# Autodesk Inventor assembly: ASY ДМФ 0100 Барабан v2.1
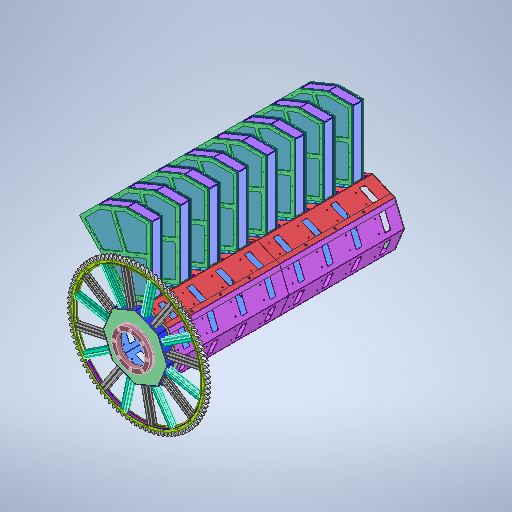
[picture p0: Inventor's stored thumbnail of the model, 512x512]
Saved by Autodesk Inventor 2025 (Build 290162010, 162A)
## iProperties
Created: 2024-04-28
Part Number: ASY ДМФ 0100 Барабан v2.1
Document SubType Name: Assembly
Designer: pokla
Author: pokla
## Documents named in this file (29)
- C:\Users\pokla\Documents\Inventor\ДФО\ДМФ\DMF-Disk-Micro-Filter\Барабан v2.1\ASY ДМФ 0100 Барабан v2.1.iam
- C:\Users\pokla\Documents\Inventor\ДФО\ДМФ\DMF-Disk-Micro-Filter\Барабан v2.1\DMF 01 21 Барабан торец НОС v2.1.ipt
- C:\Users\pokla\Documents\Inventor\ДФО\ДМФ\DMF-Disk-Micro-Filter\Барабан v2.1\DMF 01 13 Барабан Лист лев брт v2.1.ipt
- C:\Users\pokla\Documents\Inventor\ДФО\ДМФ\DMF-Disk-Micro-Filter\Барабан v2.1\DMF 01 14 Барабан Лист прав брт v2.1.ipt
- C:\Users\pokla\Documents\Inventor\ДФО\ДМФ\DMF-Disk-Micro-Filter\Барабан v2.1\DMF 01 31 Барабан Опорное кольцо НОС v2.1.ipt
- C:\Users\pokla\Documents\Inventor\ДФО\ДМФ\DMF-Disk-Micro-Filter\Барабан v2.1\DMF 01 17 опора крышки v2.1.ipt
- C:\Users\pokla\Documents\Inventor\ДФО\ДМФ\DMF-Disk-Micro-Filter\Барабан v2.1\DMF 000 размеры v2.1.ipt
- C:\Users\pokla\Documents\Inventor\ДФО\ДМФ\DMF-Disk-Micro-Filter\Барабан v2.1\DMF 01 12 Барабан усилитель v2.1.ipt
- C:\Users\pokla\Documents\Inventor\ДФО\ДМФ\DMF-Disk-Micro-Filter\Барабан v2.1\ASY DMF 010 cap v2.1.iam
- C:\Users\pokla\Documents\Inventor\ДФО\ДМФ\DMF-Disk-Micro-Filter\Барабан v2.1\DMF 01 32 Барабан Опорное кольцо КОРМА v2.1.ipt
- C:\Users\pokla\Documents\Inventor\ДФО\ДМФ\DMF-Disk-Micro-Filter\Барабан v2.1\DMF 01 22 Барабан торец КОРМА v2.1.ipt
- C:\Users\pokla\Documents\Inventor\ДФО\ДМФ\DMF-Disk-Micro-Filter\Барабан v2.1\ASY DMF filter package v2.1.iam
- C:\Users\pokla\Documents\Inventor\ДФО\ДМФ\DMF-Disk-Micro-Filter\Барабан v2.1\DMF 01 21 cylinder butt end nose.ipt
- C:\Users\pokla\Documents\Inventor\ДФО\ДМФ\DMF-Disk-Micro-Filter\Барабан v2.1\DMF 2.1 01 42 Gear way 2.ipt
- C:\Users\pokla\Documents\Inventor\ДФО\ДМФ\DMF-Disk-Micro-Filter\Барабан v2.1\DMF 2.1 01 43 Gear rim 3.ipt
- C:\Users\pokla\Documents\Inventor\ДФО\ДМФ\DMF-Disk-Micro-Filter\Барабан v2.1\DMF 2.1 01 44 Gear rim 4.ipt
- C:\Users\pokla\Documents\Inventor\ДФО\ДМФ\DMF-Disk-Micro-Filter\Барабан v2.1\DMF 2.1 01 45 Gear ring 5.ipt
- C:\Users\pokla\Documents\Inventor\ДФО\ДМФ\DMF-Disk-Micro-Filter\Барабан v2.1\DMF 2.1 01 46 Gear axis wheel 6.ipt
- C:\Users\pokla\Documents\Inventor\ДФО\ДМФ\DMF-Disk-Micro-Filter\Барабан v2.1\DMF 01 13 Барабан усилитель v2.1.ipt
- C:\Users\pokla\Documents\Inventor\ДФО\ДМФ\DMF-Disk-Micro-Filter\шестерни 06.09.2025\DMF sector big gear 2.1.ipt
- C:\Users\pokla\Documents\Inventor\ДФО\ДМФ\DMF-Disk-Micro-Filter\Барабан v2.1\DMF 01 15 drum sheet 1.ipt
- C:\Users\pokla\Documents\Inventor\ДФО\ДМФ\DMF-Disk-Micro-Filter\ДМФ 01 12 Барабан усилитель.ipt
- C:\Users\pokla\Documents\Inventor\ДФО\ДМФ\DMF-Disk-Micro-Filter\ДМФ 01 15 Барабан усилитель борта.ipt
- C:\Users\pokla\Documents\Inventor\ДФО\ДМФ\DMF-Disk-Micro-Filter\Барабан v2.1\DMF 2.1 Пластина паза маленькая.ipt
- C:\Users\pokla\Documents\Inventor\ДФО\ДМФ\DMF-Disk-Micro-Filter\Барабан v2.1\DMF 2.1 Пластина паза большая.ipt
- C:\Users\pokla\Documents\Inventor\ДФО\ДМФ\DMF-Disk-Micro-Filter\Барабан v2.1\DMF 01 14 Барабан Лист прав брт №2 v2.1.ipt
- C:\Users\pokla\Documents\Inventor\ДФО\ДМФ\DMF-Disk-Micro-Filter\Барабан v2.1\DMF 01 13 Барабан Лист лев брт №2 v2.1.ipt
- C:\Users\pokla\Documents\Inventor\ДФО\ДМФ\DMF-Disk-Micro-Filter\Барабан v2.1\ASY DMF 010 cap №2 v2.1.iam
- C:\Users\pokla\Documents\Inventor\ДФО\ДМФ\DMF-Disk-Micro-Filter\Барабан v2.1\DMF 01 17 опора крышки v2.1_CPY.ipt
## Components (125 placed, 36 different names)
1. DMF 000 размеры v2.1.ipt:1
2. DMF 01 21 Барабан торец НОС v2.1.ipt:1 — Mate:41, Flush:29, Flush:30, Mate:42, Flush:31, Flush:32, Rigid:80, Rigid:81
3. DMF 01 31 Барабан Опорное кольцо НОС v2.1.ipt:1 — Rigid:80
4. DMF 01 32 Барабан Опорное кольцо КОРМА v2.1.ipt:1 — Rigid:20
5. DMF 01 22 Барабан торец КОРМА v2.1.ipt:1 — Rigid:20, Rigid:51, Rigid:53, Mate:36, Flush:22, Flush:23, Mate:37, Flush:24, Flush:25, Mate:45, Flush:34, Flush:35
6. DMF 01 13 Барабан Лист лев брт v2.1.ipt:1 — Rigid:51, Rigid:86
7. DMF 01 14 Барабан Лист прав брт v2.1.ipt:1 — Rigid:53, Rigid:85
8. DMF 01 17 опора крышки v2.1.ipt:1 — Mate:37, Flush:24, Flush:25, Rigid:93
9. DMF 01 17 опора крышки v2.1.ipt:2 — Mate:36, Flush:22, Flush:23, Rigid:92
10. ASY DMF 010 cap v2.1.iam:1 [sub-assembly] — Mate:45, Flush:34, Flush:35, Rigid:84, Rigid:90, Rigid:91
11. DMF 01 21 cylinder butt end nose.ipt:1
12. DMF 2.1 01 45 Gear ring 5.ipt:1
13. DMF 2.1 01 46 Gear axis wheel 6.ipt:1
14. DMF 2.1 01 44 Gear rim 4.ipt:1 — Rigid:39, Rigid:40, Rigid:41
15. DMF 2.1 01 43 Gear rim 3.ipt:2 — Rigid:24, Rigid:35
16. DMF 2.1 01 43 Gear rim 3.ipt:1 — Rigid:24
17. DMF 2.1 01 43 Gear rim 3.ipt:3 — Rigid:35, Rigid:36, Rigid:39
18. DMF 2.1 01 43 Gear rim 3.ipt:4
19. DMF 2.1 01 43 Gear rim 3.ipt:5 — Rigid:36, Rigid:38, Rigid:81
20. DMF 2.1 01 43 Gear rim 3.ipt:6 — Rigid:42
21. DMF 2.1 01 43 Gear rim 3.ipt:7 — Rigid:38, Tangent:1
22. DMF 2.1 01 43 Gear rim 3.ipt:8
23. DMF 2.1 01 44 Gear rim 4.ipt:2 — Rigid:40
24. DMF 2.1 01 44 Gear rim 4.ipt:3 — Rigid:41
25. DMF 01 15 drum sheet 1.ipt:1 — Mate:41, Flush:29, Flush:30, Flush:33, Mate:43, Mate:50, Mate:51, Flush:38, Flush:39
26. DMF 01 15 drum sheet 1.ipt:2 — Mate:42, Flush:31, Flush:32, Mate:44
27. ДМФ 01 12 Барабан усилитель.ipt:2 — Rigid:56, Rigid:57, Flush:33, Mate:43, Mate:44, Rigid:89
28. ДМФ 01 15 Барабан усилитель борта.ipt:3 — Rigid:56
29. ДМФ 01 15 Барабан усилитель борта.ipt:4 — Rigid:57
30. DMF 01 14 Барабан Лист прав брт №2 v2.1:1 — Rigid:85
31. DMF 01 13 Барабан Лист лев брт №2 v2.1:1 — Rigid:86
32. ASY DMF 010 cap №2 v2.1:1 [sub-assembly] — Rigid:84, Flush:40, Mate:52, Mate:53
33. ДМФ 01 12 Барабан усилитель:3 — Flush:40, Mate:52, Mate:53, Rigid:89
34. ДМФ 01 15 Барабан усилитель борта:5
35. ДМФ 01 15 Барабан усилитель борта:6
36. DMF 01 17 опора крышки №2 v2.1:1 — Rigid:92
37. DMF 01 17 опора крышки №2 v2.1:2 — Rigid:93
38. DMF sector big gear 2.1.ipt:1 — Rigid:42
39. DMF sector big gear 2.1:2
40. DMF sector big gear 2.1:3
41. DMF sector big gear 2.1:4
42. DMF sector big gear 2.1:5
43. DMF sector big gear 2.1:6
44. DMF sector big gear 2.1:7
45. DMF sector big gear 2.1:8
46. DMF sector big gear 2.1:9
47. DMF sector big gear 2.1:10
48. DMF sector big gear 2.1:11
49. DMF sector big gear 2.1:12
50. DMF sector big gear 2.1:13
51. DMF sector big gear 2.1:14
52. DMF sector big gear 2.1:15
53. DMF sector big gear 2.1:16
54. DMF sector big gear 2.1:17
55. DMF sector big gear 2.1:18
56. DMF sector big gear 2.1:19
57. DMF sector big gear 2.1:20
58. DMF sector big gear 2.1:21
59. DMF sector big gear 2.1:22
60. DMF sector big gear 2.1:23
61. DMF sector big gear 2.1:24
62. DMF 01 13 Барабан усилитель v2.1.ipt:2 — Rigid:83, Tangent:1
63. DMF 01 12 Барабан усилитель v2.1.ipt:2 — Rigid:83, Symmetry:1, Mate:50, Flush:38
64. DMF 01 13 Барабан усилитель v2.1.ipt:1 — Rigid:82
65. DMF 01 12 Барабан усилитель v2.1.ipt:1 — Rigid:82, Symmetry:1, Mate:51, Flush:39
66. ДМФ 01 13 Барабан усилитель v2.0:3
67. DMF 01 12 Барабан усилитель v2.1:52
68. ДМФ 01 13 Барабан усилитель v2.0:4
69. DMF 01 12 Барабан усилитель v2.1:53
70. ДМФ 01 13 Барабан усилитель v2.0:5
71. DMF 01 12 Барабан усилитель v2.1:54
72. ДМФ 01 13 Барабан усилитель v2.0:6
73. DMF 01 12 Барабан усилитель v2.1:55
74. ДМФ 01 13 Барабан усилитель v2.0:7
75. DMF 01 12 Барабан усилитель v2.1:56
76. ДМФ 01 13 Барабан усилитель v2.0:8
77. DMF 01 12 Барабан усилитель v2.1:57
78. ДМФ 01 13 Барабан усилитель v2.0:9
79. DMF 01 12 Барабан усилитель v2.1:58
80. ДМФ 01 13 Барабан усилитель v2.0:10
81. DMF 01 12 Барабан усилитель v2.1:59
82. ДМФ 01 13 Барабан усилитель v2.0:11
83. DMF 01 12 Барабан усилитель v2.1:60
84. ДМФ 01 13 Барабан усилитель v2.0:12
85. DMF 01 12 Барабан усилитель v2.1:61
86. ДМФ 01 13 Барабан усилитель v2.0:13
87. DMF 01 12 Барабан усилитель v2.1:62
88. ДМФ 01 13 Барабан усилитель v2.0:14
89. DMF 01 12 Барабан усилитель v2.1:63
90. ДМФ 01 13 Барабан усилитель v2.0:15
91. DMF 01 12 Барабан усилитель v2.1:64
92. ДМФ 01 13 Барабан усилитель v2.0:16
93. DMF 01 12 Барабан усилитель v2.1:65
94. ASY DMF filter package v2.1.iam:1 [sub-assembly] — Rigid:59
95. DMF 2.1 01 42 Gear way 2.ipt:1 — Rigid:59, Rigid:91
96. DMF 2.1 Пластина паза большая:1 — Rigid:62
97. DMF 2.1 Пластина паза маленькая.ipt:1 — Rigid:62, Rigid:90
98. ASY DMF filter package v2.1:2 [sub-assembly]
99. DMF 2.1 01 42 Gear way 2:2
100. DMF 2.1 Пластина паза большая:2
101. DMF 2.1 Пластина паза маленькая:2
102. ASY DMF filter package v2.1:3 [sub-assembly]
103. DMF 2.1 01 42 Gear way 2:3
104. DMF 2.1 Пластина паза большая:3
105. DMF 2.1 Пластина паза маленькая:3
106. ASY DMF filter package v2.1:4 [sub-assembly]
107. DMF 2.1 01 42 Gear way 2:4
108. DMF 2.1 Пластина паза большая:4
109. DMF 2.1 Пластина паза маленькая:4
110. ASY DMF filter package v2.1:5 [sub-assembly]
111. DMF 2.1 01 42 Gear way 2:5
112. DMF 2.1 Пластина паза большая:5
113. DMF 2.1 Пластина паза маленькая:5
114. ASY DMF filter package v2.1:6 [sub-assembly]
115. DMF 2.1 01 42 Gear way 2:6
116. DMF 2.1 Пластина паза большая:6
117. DMF 2.1 Пластина паза маленькая:6
118. ASY DMF filter package v2.1:7 [sub-assembly]
119. DMF 2.1 01 42 Gear way 2:7
120. DMF 2.1 Пластина паза большая:7
121. DMF 2.1 Пластина паза маленькая:7
122. ASY DMF filter package v2.1:8 [sub-assembly]
123. DMF 2.1 01 42 Gear way 2:8
124. DMF 2.1 Пластина паза большая:8
125. DMF 2.1 Пластина паза маленькая:8
## Component patterns: (24 elements, first: DMF sector big gear 2.1.ipt:1), (8 elements, first: DMF 01 13 Барабан усилитель v2.1.ipt:2 + DMF 01 12 Барабан усилитель v2.1.ipt:2 + DMF 01 13 Барабан усилитель v2.1.ipt:1 + DMF 01 12 Барабан усилитель v2.1.ipt:1), (8 elements, first: ASY DMF filter package v2.1.iam:1 + DMF 2.1 01 42 Gear way 2.ipt:1 + DMF 2.1 Пластина паза большая:1 + DMF 2.1 Пластина паза маленькая.ipt:1)
## Relationships (59: WeldJoint 32, Flush 14, Mate 11, Symmetry 1, Tangent 1)
- Rigid:20 [WeldJoint]: DMF 01 32 Барабан Опорное кольцо КОРМА v2.1.ipt:1 ↔ DMF 01 22 Барабан торец КОРМА v2.1.ipt:1
- Rigid:24 [WeldJoint] (25 mm): DMF 2.1 01 43 Gear rim 3.ipt:2 ↔ DMF 2.1 01 43 Gear rim 3.ipt:1
- [WeldJoint] (25 mm): DMF 2.1 01 43 Gear rim 3.ipt:3 ↔ DMF 2.1 01 43 Gear rim 3.ipt:4
- [WeldJoint] (25 mm): DMF 2.1 01 43 Gear rim 3.ipt:5 ↔ DMF 2.1 01 43 Gear rim 3.ipt:6
- Rigid:35 [WeldJoint]: DMF 2.1 01 43 Gear rim 3.ipt:2 ↔ DMF 2.1 01 43 Gear rim 3.ipt:3
- Rigid:36 [WeldJoint]: DMF 2.1 01 43 Gear rim 3.ipt:3 ↔ DMF 2.1 01 43 Gear rim 3.ipt:5
- [WeldJoint] (25 mm): DMF 2.1 01 43 Gear rim 3.ipt:7 ↔ DMF 2.1 01 43 Gear rim 3.ipt:8
- Rigid:38 [WeldJoint]: DMF 2.1 01 43 Gear rim 3.ipt:5 ↔ DMF 2.1 01 43 Gear rim 3.ipt:7
- Rigid:39 [WeldJoint]: DMF 2.1 01 44 Gear rim 4.ipt:1 ↔ DMF 2.1 01 43 Gear rim 3.ipt:3
- Rigid:40 [WeldJoint]: DMF 2.1 01 44 Gear rim 4.ipt:1 ↔ DMF 2.1 01 44 Gear rim 4.ipt:2
- Rigid:41 [WeldJoint]: DMF 2.1 01 44 Gear rim 4.ipt:1 ↔ DMF 2.1 01 44 Gear rim 4.ipt:3
- Rigid:42 [WeldJoint]: DMF 2.1 01 43 Gear rim 3.ipt:6 ↔ DMF sector big gear 2.1.ipt:1
- Rigid:51 [WeldJoint]: DMF 01 22 Барабан торец КОРМА v2.1.ipt:1 ↔ DMF 01 13 Барабан Лист лев брт v2.1.ipt:1
- Rigid:53 [WeldJoint]: DMF 01 22 Барабан торец КОРМА v2.1.ipt:1 ↔ DMF 01 14 Барабан Лист прав брт v2.1.ipt:1
- Mate:36: DMF 01 22 Барабан торец КОРМА v2.1.ipt:1 ↔ DMF 01 17 опора крышки v2.1.ipt:2
- Flush:22 (2 mm): DMF 01 22 Барабан торец КОРМА v2.1.ipt:1 ↔ DMF 01 17 опора крышки v2.1.ipt:2
- Flush:23 (2 mm): DMF 01 22 Барабан торец КОРМА v2.1.ipt:1 ↔ DMF 01 17 опора крышки v2.1.ipt:2
- Mate:37: DMF 01 22 Барабан торец КОРМА v2.1.ipt:1 ↔ DMF 01 17 опора крышки v2.1.ipt:1
- Flush:24 (2 mm): DMF 01 22 Барабан торец КОРМА v2.1.ipt:1 ↔ DMF 01 17 опора крышки v2.1.ipt:1
- Flush:25 (2 mm): DMF 01 22 Барабан торец КОРМА v2.1.ipt:1 ↔ DMF 01 17 опора крышки v2.1.ipt:1
- Rigid:56 [WeldJoint]: ДМФ 01 12 Барабан усилитель.ipt:2 ↔ ДМФ 01 15 Барабан усилитель борта.ipt:3
- Rigid:57 [WeldJoint]: ДМФ 01 12 Барабан усилитель.ipt:2 ↔ ДМФ 01 15 Барабан усилитель борта.ipt:4
- Mate:41: DMF 01 21 Барабан торец НОС v2.1.ipt:1 ↔ DMF 01 15 drum sheet 1.ipt:1
- Flush:29: DMF 01 21 Барабан торец НОС v2.1.ipt:1 ↔ DMF 01 15 drum sheet 1.ipt:1
- Flush:30: DMF 01 21 Барабан торец НОС v2.1.ipt:1 ↔ DMF 01 15 drum sheet 1.ipt:1
- Mate:42: DMF 01 21 Барабан торец НОС v2.1.ipt:1 ↔ DMF 01 15 drum sheet 1.ipt:2
- Flush:31: DMF 01 21 Барабан торец НОС v2.1.ipt:1 ↔ DMF 01 15 drum sheet 1.ipt:2
- Flush:32: DMF 01 21 Барабан торец НОС v2.1.ipt:1 ↔ DMF 01 15 drum sheet 1.ipt:2
- Flush:33: DMF 01 15 drum sheet 1.ipt:1 ↔ ДМФ 01 12 Барабан усилитель.ipt:2
- Mate:43: DMF 01 15 drum sheet 1.ipt:1 ↔ ДМФ 01 12 Барабан усилитель.ipt:2
- Mate:44: DMF 01 15 drum sheet 1.ipt:2 ↔ ДМФ 01 12 Барабан усилитель.ipt:2
- Mate:45: DMF 01 22 Барабан торец КОРМА v2.1.ipt:1 ↔ ASY DMF 010 cap v2.1.iam:1
- Flush:34: DMF 01 22 Барабан торец КОРМА v2.1.ipt:1 ↔ ASY DMF 010 cap v2.1.iam:1
- Flush:35: DMF 01 22 Барабан торец КОРМА v2.1.ipt:1 ↔ ASY DMF 010 cap v2.1.iam:1
- Rigid:59 [WeldJoint] (5 mm): ASY DMF filter package v2.1.iam:1 ↔ DMF 2.1 01 42 Gear way 2.ipt:1
- Rigid:62 [WeldJoint]: DMF 2.1 Пластина паза большая:1 ↔ DMF 2.1 Пластина паза маленькая.ipt:1
- Rigid:80 [WeldJoint]: DMF 01 21 Барабан торец НОС v2.1.ipt:1 ↔ DMF 01 31 Барабан Опорное кольцо НОС v2.1.ipt:1
- Rigid:81 [WeldJoint] (-20.5 mm): DMF 01 21 Барабан торец НОС v2.1.ipt:1 ↔ DMF 2.1 01 43 Gear rim 3.ipt:5
- Rigid:82 [WeldJoint]: DMF 01 13 Барабан усилитель v2.1.ipt:1 ↔ DMF 01 12 Барабан усилитель v2.1.ipt:1
- Rigid:83 [WeldJoint]: DMF 01 13 Барабан усилитель v2.1.ipt:2 ↔ DMF 01 12 Барабан усилитель v2.1.ipt:2
- Symmetry:1: DMF 01 12 Барабан усилитель v2.1.ipt:2 ↔ DMF 01 12 Барабан усилитель v2.1.ipt:1
- Mate:50: DMF 01 15 drum sheet 1.ipt:1 ↔ DMF 01 12 Барабан усилитель v2.1.ipt:2
- Mate:51: DMF 01 15 drum sheet 1.ipt:1 ↔ DMF 01 12 Барабан усилитель v2.1.ipt:1
- Flush:38 (15 mm): DMF 01 15 drum sheet 1.ipt:1 ↔ DMF 01 12 Барабан усилитель v2.1.ipt:2
- Flush:39 (15 mm): DMF 01 15 drum sheet 1.ipt:1 ↔ DMF 01 12 Барабан усилитель v2.1.ipt:1
- Tangent:1: DMF 2.1 01 43 Gear rim 3.ipt:7 ↔ DMF 01 13 Барабан усилитель v2.1.ipt:2
- Rigid:84 [WeldJoint]: ASY DMF 010 cap v2.1.iam:1 ↔ ASY DMF 010 cap №2 v2.1:1
- Rigid:85 [WeldJoint]: DMF 01 14 Барабан Лист прав брт v2.1.ipt:1 ↔ DMF 01 14 Барабан Лист прав брт №2 v2.1:1
- Rigid:86 [WeldJoint]: DMF 01 13 Барабан Лист лев брт v2.1.ipt:1 ↔ DMF 01 13 Барабан Лист лев брт №2 v2.1:1
- [WeldJoint]: ДМФ 01 12 Барабан усилитель:3 ↔ ДМФ 01 15 Барабан усилитель борта:5
- [WeldJoint]: ДМФ 01 12 Барабан усилитель:3 ↔ ДМФ 01 15 Барабан усилитель борта:6
- Flush:40: ASY DMF 010 cap №2 v2.1:1 ↔ ДМФ 01 12 Барабан усилитель:3
- Mate:52: ASY DMF 010 cap №2 v2.1:1 ↔ ДМФ 01 12 Барабан усилитель:3
- Mate:53: ASY DMF 010 cap №2 v2.1:1 ↔ ДМФ 01 12 Барабан усилитель:3
- Rigid:89 [WeldJoint]: ДМФ 01 12 Барабан усилитель.ipt:2 ↔ ДМФ 01 12 Барабан усилитель:3
- Rigid:90 [WeldJoint] (-48.5 mm): ASY DMF 010 cap v2.1.iam:1 ↔ DMF 2.1 Пластина паза маленькая.ipt:1
- Rigid:91 [WeldJoint]: ASY DMF 010 cap v2.1.iam:1 ↔ DMF 2.1 01 42 Gear way 2.ipt:1
- Rigid:92 [WeldJoint]: DMF 01 17 опора крышки v2.1.ipt:2 ↔ DMF 01 17 опора крышки №2 v2.1:1
- Rigid:93 [WeldJoint]: DMF 01 17 опора крышки v2.1.ipt:1 ↔ DMF 01 17 опора крышки №2 v2.1:2
## Named parameters: d314_d251 = 25 mm, d315_d251 = 25 mm, d318_d251 = 25 mm, d460_d378 = 0 mm, d461_d379 = 0 mm
